# Autodesk Inventor assembly: Bottom Roller
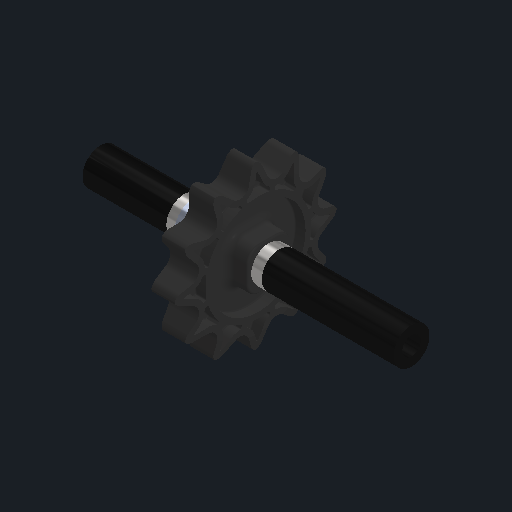
[picture p0: Inventor's stored thumbnail of the model, 512x512]
Saved by Autodesk Inventor 2025 (Build 290162000, 162)
## iProperties
Created: 2024-12-25
Part Number: Bottom Roller
Document SubType Name: Assembly
Designer: Averey Ku
Author: Averey Ku
## Documents named in this file (11)
- D:\VEX\High Stakes\CAD\V4\Conveyer\Bottom Roller.iam
- D:\VEX\High Stakes\CAD\ROBOPROS-CAD-Inventor\Motion\Sprockets\9P Sprocket\9P 12T Sprocket, No Insert.iam
- D:\VEX\High Stakes\CAD\ROBOPROS-CAD-Inventor\Motion\Sprockets\9P Sprocket.iam
- D:\VEX\High Stakes\CAD\ROBOPROS-CAD-Inventor\Motion\Shaft LS\Shaft Collar ipts\Shaft Collar Set Screw.ipt
- D:\VEX\High Stakes\CAD\ROBOPROS-CAD-Inventor\Motion\Spacers\Washer Steel\SWasher .375 OD x .015625.ipt
- D:\VEX\High Stakes\CAD\ROBOPROS-CAD-Inventor\Motion\Spacers\Washer Steel.ipt
- D:\VEX\High Stakes\CAD\ROBOPROS-CAD-Inventor\Motion\Spacers\Washer Steel\SWasher .375 OD x .031250.ipt
- D:\VEX\High Stakes\CAD\ROBOPROS-CAD-Inventor\Motion\Spacers\Washer Steel\SWasher .375 OD x .062500.ipt
- D:\VEX\High Stakes\CAD\ROBOPROS-CAD-Inventor\Motion\Spacers\Spacer Nylon .375 OD\NSpacer .375 OD x .500.ipt
- D:\VEX\High Stakes\CAD\ROBOPROS-CAD-Inventor\Motion\Spacers\Spacer Nylon .375 OD.ipt
- D:\VEX\High Stakes\CAD\ROBOPROS-CAD-Inventor\Motion\Spacers\Spacer Nylon .375 OD\NSpacer .375 OD x .375.ipt
## Components (13 placed, 7 different names)
1. 9P 12T Sprocket, No Insert:1 [sub-assembly] — Insert:1, Insert:14
2. Shaft Collar Set Screw:1 — Insert:1, Insert:4
3. SWasher .375 OD x .015625:1 — Insert:2, Insert:7
4. SWasher .375 OD x .031250:2 — Insert:2, Insert:3
5. SWasher .375 OD x .062500:3 — Insert:3, Insert:4
6. NSpacer .375 OD x .500:1 — Insert:5, Insert:7
7. NSpacer .375 OD x .375:3 — Insert:5
8. SWasher .375 OD x .015625:4
9. SWasher .375 OD x .031250:5
10. SWasher .375 OD x .062500:6 — Insert:14
11. NSpacer .375 OD x .500:4
12. NSpacer .375 OD x .375:6 — Insert:13
13. NSpacer .375 OD x .500:7 — Insert:13
## Relationships (12: Insert 12)
- Insert:1: 9P 12T Sprocket, No Insert:1 ↔ Shaft Collar Set Screw:1
- Insert:2: SWasher .375 OD x .015625:1 ↔ SWasher .375 OD x .031250:2
- Insert:3: SWasher .375 OD x .031250:2 ↔ SWasher .375 OD x .062500:3
- Insert:4: Shaft Collar Set Screw:1 ↔ SWasher .375 OD x .062500:3
- Insert:5: NSpacer .375 OD x .500:1 ↔ NSpacer .375 OD x .375:3
- Insert:7: SWasher .375 OD x .015625:1 ↔ NSpacer .375 OD x .500:1
- [Insert]: SWasher .375 OD x .015625:4 ↔ SWasher .375 OD x .031250:5
- [Insert]: SWasher .375 OD x .031250:5 ↔ SWasher .375 OD x .062500:6
- [Insert]: NSpacer .375 OD x .500:4 ↔ NSpacer .375 OD x .375:6
- [Insert]: SWasher .375 OD x .015625:4 ↔ NSpacer .375 OD x .500:4
- Insert:13: NSpacer .375 OD x .375:6 ↔ NSpacer .375 OD x .500:7
- Insert:14: 9P 12T Sprocket, No Insert:1 ↔ SWasher .375 OD x .062500:6
## Named parameters: d9_d3 = 0 mm, d10_d4 = 0 mm, d11_d6 = 0 mm, d13_d8 = 0 mm
